# Autodesk Inventor assembly: 2ndAxis
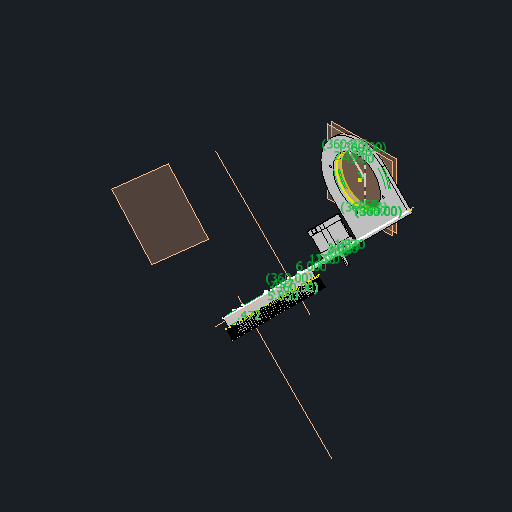
[picture p0: Inventor's stored thumbnail of the model, 512x512]
Saved by Autodesk Inventor 2024 (Build 280153000, 153)
## iProperties
Created: 2023-10-21
Part Number: 2ndAxis
Document SubType Name: Assembly
Designer: range
Author: range
## Documents named in this file (7)
- C:\Users\range\CodingProjects\C-AAM\CAD\V1\Parts\2ndAxis.iam
- C:\Users\range\CodingProjects\C-AAM\CAD\V1\Parts\TopSpacer.ipt
- C:\Users\range\CodingProjects\C-AAM\CAD\V1\Parts\AxisBoard.ipt
- C:\Users\range\CodingProjects\C-AAM\CAD\V1\Parts\SideBoard.ipt
- C:\Users\range\CodingProjects\C-AAM\CAD\V1\Parts\LazySusan.iam
- C:\Users\range\CodingProjects\C-AAM\CAD\V1\LargePitchAssembly.iam
- C:\Users\range\CodingProjects\C-AAM\CAD\V1\6627T91_Stepper Motor\6627T91_Stepper Motor.ipt
## Components (6 placed, 6 different names)
1. TopSpacer:1 — Flush:1, Flush:2
2. AxisBoard:1 — Flush:1, Flush:2, Flush:3, Flush:4, Angle:1, Angle:3, Flush:5, Flush:6
3. SideBoard:1 — Flush:3, Flush:4, Mate:2, Angle:2, Mate:10, Mate:11, Flush:5, Flush:6
4. LazySusan:1 [sub-assembly] — Mate:2, Mate:3, Mate:4, Angle:2, Mate:7, Mate:8, Mate:9
5. LargePitchAssembly:1 [sub-assembly] — Mate:7, Mate:8, Mate:9
6. 6627T91_Stepper Motor:1 — Mate:10, Angle:3, Mate:11
## Relationships (19: Mate 10, Flush 6, Angle 3)
- Flush:1: TopSpacer:1 ↔ AxisBoard:1
- Flush:2: TopSpacer:1 ↔ AxisBoard:1
- Flush:3: AxisBoard:1 ↔ SideBoard:1
- Flush:4: AxisBoard:1 ↔ SideBoard:1
- Mate:2: SideBoard:1 ↔ LazySusan:1
- Mate:3: LazySusan:1
- Mate:4: LazySusan:1
- Mate:5
- Mate:6
- Angle:1 (0 deg): AxisBoard:1
- Angle:2 (180 deg): SideBoard:1 ↔ LazySusan:1
- Mate:7: LazySusan:1 ↔ LargePitchAssembly:1
- Mate:8: LazySusan:1 ↔ LargePitchAssembly:1
- Mate:9: LazySusan:1 ↔ LargePitchAssembly:1
- Mate:10: SideBoard:1 ↔ 6627T91_Stepper Motor:1
- Angle:3 (0 deg): AxisBoard:1 ↔ 6627T91_Stepper Motor:1
- Mate:11: SideBoard:1 ↔ 6627T91_Stepper Motor:1
- Flush:5: AxisBoard:1 ↔ SideBoard:1
- Flush:6: AxisBoard:1 ↔ SideBoard:1
